# Autodesk Inventor assembly: Gallows
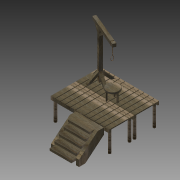
[picture p0: Inventor's stored thumbnail of the model, 180x180]
Saved by Autodesk Inventor 2015 (Build 190159000, 159)
## iProperties
Created: 2016-10-21
Part Number: Gallows
Document SubType Name: Assembly
Designer: kelloggcha95
Author: kelloggcha95
## Documents named in this file (6)
- Z:\Gallows.iam
- Z:\deck.ipt
- Z:\Stairs.ipt
- Z:\Gallows 1.ipt
- Z:\three.ipt
- Z:\Noose.ipt
## Components (8 placed, 5 different names)
1. deck:1 — Mate:1, Mate:2
2. deck:2 — Mate:1, Mate:3, Mate:4
3. deck:3 — Mate:2, Mate:5
4. deck:4 — Mate:3, Mate:6
5. Stairs:1 — Mate:4
6. Gallows 1:1 — Mate:5, Mate:7
7. three:1 — Mate:6
8. Noose:1 — Mate:7
## Relationships (7: Mate 7)
- Mate:1: deck:1 ↔ deck:2
- Mate:2: deck:1 ↔ deck:3
- Mate:3: deck:2 ↔ deck:4
- Mate:4: deck:2 ↔ Stairs:1
- Mate:5: deck:3 ↔ Gallows 1:1
- Mate:6: deck:4 ↔ three:1
- Mate:7: Gallows 1:1 ↔ Noose:1
